# Autodesk Inventor assembly: circular polarizer
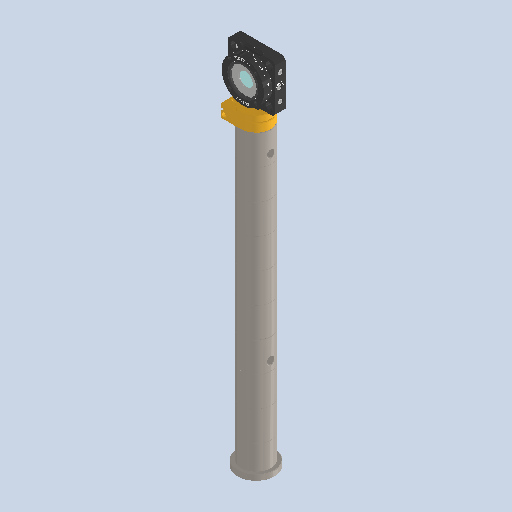
[picture p0: Inventor's stored thumbnail of the model, 512x512]
Saved by Autodesk Inventor 2026.1 (Build 301233000, 233)
## iProperties
Created: 2025-06-02
Part Number: circular polarizer
Document SubType Name: Assembly
Designer: Julian
Author: Julian
## Documents named in this file (6)
- C:\Users\user\Desktop\setup_inventor_2025\circular polarizer\circular polarizer.iam
- C:\Users\user\Desktop\setup_inventor_2025\circular polarizer\Newport-M-PS-4-1.ipt
- C:\Users\user\Desktop\setup_inventor_2025\circular polarizer\Newport-M-PS-6E-.ipt
- C:\Users\user\Desktop\setup_inventor_2025\circular polarizer\Newpor-M-PS-KF.ipt
- C:\Users\user\Desktop\setup_inventor_2025\circular polarizer\AQWP05M-980.ipt
- C:\Users\user\Desktop\setup_inventor_2025\circular polarizer\CRM1T_M.ipt
## Components (5 placed, 5 different names)
1. Newport-M-PS-4-1:1 — Passend:4, Passend:7
2. Newport-M-PS-6E-:1 — Passend:3, Passend:4, Passend:6, Passend:7
3. Newpor-M-PS-KF:1 — Passend:2, Passend:3, Passend:5, Passend:6
4. AQWP05M-980:1 — Passend:1, Fluchtend:1
5. CRM1T_M:1 — Passend:1, Fluchtend:1, Passend:2, Passend:5
## Relationships (8: Mate 7, Flush 1)
- Passend:1 [Mate]: AQWP05M-980:1 ↔ CRM1T_M:1
- Fluchtend:1 [Flush] (-2 mm): AQWP05M-980:1 ↔ CRM1T_M:1
- Passend:2 [Mate]: Newpor-M-PS-KF:1 ↔ CRM1T_M:1
- Passend:3 [Mate]: Newport-M-PS-6E-:1 ↔ Newpor-M-PS-KF:1
- Passend:4 [Mate]: Newport-M-PS-4-1:1 ↔ Newport-M-PS-6E-:1
- Passend:5 [Mate]: Newpor-M-PS-KF:1 ↔ CRM1T_M:1
- Passend:6 [Mate]: Newport-M-PS-6E-:1 ↔ Newpor-M-PS-KF:1
- Passend:7 [Mate]: Newport-M-PS-4-1:1 ↔ Newport-M-PS-6E-:1
